# Autodesk Inventor assembly: Assembly_Cube_Dichroic_Beamsplitter_multi_motorized_revolver_25x35_v3
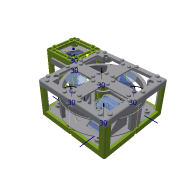
[picture p0: Inventor's stored thumbnail of the model, 180x180]
Saved by Autodesk Inventor 2019.4 (Build 234330000, 330)
## iProperties
Created: 2021-09-13
Part Number: Assembly_Cube_Dichroic_Beamsplitter_multi_motorized_revolver_25x35_v3
Document SubType Name: Assembly
Designer: diederichbenedict
Mass: 158.455 g
Surface Area: 1131.2 cm^2
Volume: 156.246 cm^3
Density: 1.01414 g/cm^3
Author: diederichbenedict
## Documents named in this file (10)
- C:\Users\diederichbenedict\Dropbox\Dokumente\Promotion\PROJECTS\UC2\02_CAD\INVENTOR\uc2_v3\Assembly_Cube_Dichroic_Beamsplitter_multi_motorized_revolver_25x35_v3.iam
- C:\Users\diederichbenedict\Dropbox\Dokumente\Promotion\PROJECTS\UC2\02_CAD\INVENTOR\uc2_v3\10_Cube_1x1_IM.ipt
- C:\Users\diederichbenedict\Dropbox\Dokumente\Promotion\PROJECTS\UC2\02_CAD\INVENTOR\uc2_v3\30_Cube_Insert_Filter_Revolver_Base_v3.ipt
- C:\Users\diederichbenedict\Dropbox\Dokumente\Promotion\PROJECTS\UC2\02_CAD\INVENTOR\uc2_v3\00_ballbearing_8mm.ipt
- C:\Users\diederichbenedict\Dropbox\Dokumente\Promotion\PROJECTS\UC2\02_CAD\INVENTOR\uc2_v3\30_Cube_Insert_Filter_Revolver_Wheel_v3.ipt
- C:\Users\diederichbenedict\Dropbox\Dokumente\Promotion\PROJECTS\UC2\02_CAD\INVENTOR\uc2_v3\30_Cube_Insert_Filter_Revolver_Filters_v3.iam
- C:\Users\diederichbenedict\Dropbox\Dokumente\Promotion\PROJECTS\UC2\02_CAD\INVENTOR\uc2_v3\30_Cube_Insert_Filter_Revolver_Wheel_Lid_v3.ipt
- C:\Users\diederichbenedict\Dropbox\Dokumente\Promotion\PROJECTS\UC2\02_CAD\INVENTOR\uc2_v3\30_Cube_Insert_Filter_Revolver_Lid.ipt
- C:\Users\diederichbenedict\Dropbox\Dokumente\Promotion\PROJECTS\UC2\02_CAD\INVENTOR\uc2_v3\30_Cube_Insert_Filter_Revolver_Wheel_centerring_v3.ipt
- C:\Users\diederichbenedict\Dropbox\Dokumente\Promotion\PROJECTS\UC2\02_CAD\INVENTOR\uc2_v3\Assembly_Cube_28byi_Motor_v3.iam
## Components (20 placed, 9 different names)
1. 30_Cube_Insert_Filter_Revolver_Wheel_v3:1 — Mate:18, Mate:19, Angle:3, Mate:26, Flush:10, Flush:11, Mate:30
2. 30_Cube_Insert_Filter_Revolver_Wheel_Lid_v3:1 — Mate:26
3. 30_Cube_Insert_Filter_Revolver_Lid:1 — Flush:8, Flush:9, Mate:27, Mate:28
4. 30_Cube_Insert_Filter_Revolver_Wheel_centerring_v3:1 — Flush:10, Flush:11
5. Assembly_Cube_28byi_Motor_v3:1 [sub-assembly] — Mate:28, Flush:12, Flush:13
6. 10_Cube_1x1_IM:1 — Mate:10, Mate:11, Mate:12
7. 30_Cube_Insert_Filter_Revolver_Base_v3:1 — Flush:1, Mate:13, Mate:14, Insert:1
8. 00_ballbearing_8mm:1 — Insert:1
9. 10_Cube_1x1_IM:2 — Mate:29, Flush:14
10. 30_Cube_Insert_Filter_Revolver_Base_v3:2
11. 00_ballbearing_8mm:2
12. 10_Cube_1x1_IM:3 — Flush:1, Mate:13, Mate:14
13. 30_Cube_Insert_Filter_Revolver_Base_v3:3
14. 00_ballbearing_8mm:3
15. 10_Cube_1x1_IM:4 — Mate:18, Flush:8, Flush:9, Mate:27, Flush:12, Flush:13
16. 30_Cube_Insert_Filter_Revolver_Base_v3:4 — Mate:19
17. 00_ballbearing_8mm:4
18. 30_Cube_Insert_Filter_Revolver_Filters_v3:1 [sub-assembly] — Mate:29, Flush:14, Mate:30
19. 30_Cube_Insert_Filter_Revolver_Filters_v3:2 [sub-assembly]
20. 30_Cube_Insert_Filter_Revolver_Filters_v3:3 [sub-assembly]
## Component patterns: (4 elements, first: 10_Cube_1x1_IM:1 + 30_Cube_Insert_Filter_Revolver_Base_v3:1 + 00_ballbearing_8mm:1), (3 elements, first: 30_Cube_Insert_Filter_Revolver_Filters_v3:1)
## Relationships (22: Mate 12, Flush 8, Insert 1, Angle 1)
- Mate:10: 10_Cube_1x1_IM:1
- Mate:11: 10_Cube_1x1_IM:1
- Mate:12: 10_Cube_1x1_IM:1
- Flush:1: 30_Cube_Insert_Filter_Revolver_Base_v3:1 ↔ 10_Cube_1x1_IM:3
- Mate:13: 30_Cube_Insert_Filter_Revolver_Base_v3:1 ↔ 10_Cube_1x1_IM:3
- Mate:14: 30_Cube_Insert_Filter_Revolver_Base_v3:1 ↔ 10_Cube_1x1_IM:3
- Insert:1: 30_Cube_Insert_Filter_Revolver_Base_v3:1 ↔ 00_ballbearing_8mm:1
- Mate:18: 30_Cube_Insert_Filter_Revolver_Wheel_v3:1 ↔ 10_Cube_1x1_IM:4
- Mate:19 (0.5 mm): 30_Cube_Insert_Filter_Revolver_Wheel_v3:1 ↔ 30_Cube_Insert_Filter_Revolver_Base_v3:4
- Angle:3 (90 deg): 30_Cube_Insert_Filter_Revolver_Wheel_v3:1
- Mate:26: 30_Cube_Insert_Filter_Revolver_Wheel_v3:1 ↔ 30_Cube_Insert_Filter_Revolver_Wheel_Lid_v3:1
- Flush:8: 30_Cube_Insert_Filter_Revolver_Lid:1 ↔ 10_Cube_1x1_IM:4
- Flush:9: 30_Cube_Insert_Filter_Revolver_Lid:1 ↔ 10_Cube_1x1_IM:4
- Mate:27: 30_Cube_Insert_Filter_Revolver_Lid:1 ↔ 10_Cube_1x1_IM:4
- Flush:10: 30_Cube_Insert_Filter_Revolver_Wheel_v3:1 ↔ 30_Cube_Insert_Filter_Revolver_Wheel_centerring_v3:1
- Flush:11: 30_Cube_Insert_Filter_Revolver_Wheel_v3:1 ↔ 30_Cube_Insert_Filter_Revolver_Wheel_centerring_v3:1
- Mate:28: 30_Cube_Insert_Filter_Revolver_Lid:1 ↔ Assembly_Cube_28byi_Motor_v3:1
- Flush:12: Assembly_Cube_28byi_Motor_v3:1 ↔ 10_Cube_1x1_IM:4
- Flush:13: Assembly_Cube_28byi_Motor_v3:1 ↔ 10_Cube_1x1_IM:4
- Mate:29 (2.5 mm): 10_Cube_1x1_IM:2 ↔ 30_Cube_Insert_Filter_Revolver_Filters_v3:1
- Flush:14 (3.5 mm): 10_Cube_1x1_IM:2 ↔ 30_Cube_Insert_Filter_Revolver_Filters_v3:1
- Mate:30: 30_Cube_Insert_Filter_Revolver_Wheel_v3:1 ↔ 30_Cube_Insert_Filter_Revolver_Filters_v3:1
